# Autodesk Inventor assembly: WeldDemo
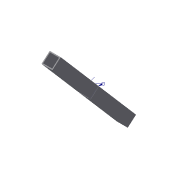
[picture p0: Inventor's stored thumbnail of the model, 180x180]
Saved by Autodesk Inventor 2017 (Build 210142000, 142)
## iProperties
Created: 2017-03-29
Part Number: WeldDemo
Document SubType Name: Weldment
Designer: krosie
Weld Material: Welded Aluminum-6061
Author: krosie
## Documents named in this file (2)
- C:\Users\krosie\Google Drive\HERA\hera-cad\feed\FeedHoopWelding\WeldDemo.iam
- C:\Users\krosie\Google Drive\HERA\hera-cad\feed\FeedHoopWelding\WeldingDemo.ipt
## Components (2 placed, 1 different names)
1. WeldingDemo:1 — Angle:1, Mate:1, Angle:2, Flush:1
2. WeldingDemo:2 — Angle:1, Mate:1, Angle:2, Flush:1
## Relationships (4: Angle 2, Mate 1, Flush 1)
- Angle:1 (0 deg): WeldingDemo:1 ↔ WeldingDemo:2
- Mate:1: WeldingDemo:1 ↔ WeldingDemo:2
- Angle:2 (0 deg): WeldingDemo:1 ↔ WeldingDemo:2
- Flush:1: WeldingDemo:1 ↔ WeldingDemo:2
